# Autodesk Inventor assembly: 00_002_SINGLE_LEG_R1
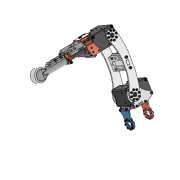
[picture p0: Inventor's stored thumbnail of the model, 180x180]
Saved by Autodesk Inventor 2021.2 (Build 252289000, 289)
## iProperties
Created: 2020-04-27
Part Number: 00_002_SINGLE_LEG_R1
Document SubType Name: Assembly
Designer: y6tada
Mass: 223.026 g
Surface Area: 749.532 cm^2
Volume: 137.086 cm^3
Density: 1.6269 g/cm^3
Author: y6tada
## Documents named in this file (4)
- C:\Workspace\HaptHexa\Hardware\Inventor\00_002_SINGLE_LEG_R1.iam
- C:\Workspace\HaptHexa\Hardware\Inventor\00_003_COXA_R1.iam
- C:\Workspace\HaptHexa\Hardware\Inventor\00_005_TIBIA_R1.iam
- C:\Workspace\HaptHexa\Hardware\Inventor\00_004_FEMUR_R1.iam
## Components (3 placed, 3 different names)
1. _Coxa:1 [sub-assembly] — Angle:1
2. 00_005_TIBIA_R1:1 [sub-assembly] — Angle:2
3. 00_004_FEMUR_R1:1 [sub-assembly] — Angle:1, Angle:2
## Relationships (4: Insert 2, Angle 2)
- [Insert]: _Coxa:1 ↔ 00_004_FEMUR_R1:1
- [Insert]: 00_005_TIBIA_R1:1 ↔ 00_004_FEMUR_R1:1
- Angle:1 (0 deg): _Coxa:1 ↔ 00_004_FEMUR_R1:1
- Angle:2 (-90 deg): 00_005_TIBIA_R1:1 ↔ 00_004_FEMUR_R1:1
## Named parameters: femur_angle = 10 deg, tibia_angle = 80 deg
